# Autodesk Inventor assembly: joint4
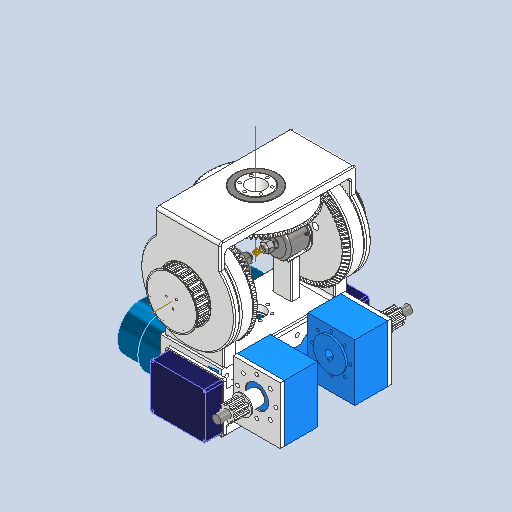
[picture p0: Inventor's stored thumbnail of the model, 512x512]
Saved by Autodesk Inventor 2025.3 (Build 293356030, 356C)
## iProperties
Created: 2025-08-31
Part Number: joint4
Document SubType Name: Assembly
Designer: MSI
Mass: 17943.2 g
Surface Area: 11658.9 cm^2
Volume: 6898.44 cm^3
Density: 2.60106 g/cm^3
Author: MSI
## Documents named in this file (16)
- C:\Users\MSI\Desktop\Project\3. 로봇팔\Robot Arm Model\Robot_Arm_6_v1\joint3.iam
- C:\Users\MSI\Desktop\Project\3. 로봇팔\Robot Arm Model\Robot_Arm_6_v1\base.ipt
- C:\Users\MSI\Desktop\Project\3. 로봇팔\Robot Arm Model\Robot_Arm_6_v1\frame.ipt
- C:\Users\MSI\Desktop\Project\3. 로봇팔\Robot Arm Model\Robot_Arm_6_v1\miter_gear_center.ipt
- C:\Users\MSI\Desktop\Project\3. 로봇팔\Robot Arm Model\Robot_Arm_6_v1\encoder.ipt
- C:\Users\MSI\Desktop\Project\3. 로봇팔\Robot Arm Model\Robot_Arm_6_v1\joint3_meteor.iam
- C:\Users\MSI\Desktop\Project\3. 로봇팔\Robot Arm Model\Robot_Arm_6_v1\encoder_frame.ipt
- C:\Users\MSI\Desktop\Project\3. 로봇팔\Robot Arm Model\Robot_Arm_6_v1\miter_gear_left_axis.ipt
- C:\Users\MSI\Desktop\Project\3. 로봇팔\Robot Arm Model\Robot_Arm_6_v1\miter_gear_right_axis.ipt
- C:\Users\MSI\Desktop\Project\3. 로봇팔\Robot Arm Model\Robot_Arm_6_v1\motor.iam
- C:\Users\MSI\Desktop\Project\3. 로봇팔\Robot Arm Model\Robot_Arm_6_v1\C-E6700ZZ_Autodesk_Inventor_2024_20250921\C-E6700ZZ.ipt
- C:\Users\MSI\Desktop\Project\3. 로봇팔\Robot Arm Model\Robot_Arm_6_v1\C-E6810ZZ_Autodesk_Inventor_2024_20250921\C-E6810ZZ.ipt
- C:\Users\MSI\Desktop\Project\3. 로봇팔\Robot Arm Model\Robot_Arm_6_v1\NTN_GS81110OuterRings\GS81110Outer Rings.ipt
- C:\Users\MSI\Desktop\Project\3. 로봇팔\Robot Arm Model\Robot_Arm_6_v1\belt_axis.ipt
- C:\Users\MSI\Desktop\Project\3. 로봇팔\Robot Arm Model\Robot_Arm_6_v1\joint3_belt_pulley_2.ipt
- C:\Users\MSI\Desktop\Project\3. 로봇팔\Robot Arm Model\Robot_Arm_6_v1\joint3_belt_pulley_1.ipt
## Components (23 placed, 14 different names)
1. motor:1 [sub-assembly] — 강체:24, 강체:36, 강체:37
2. base:1 — 회전:1, 강체:17, 강체:19, 강체:24, 강체:25, 강체:26
3. frame:1 — 회전:1, 회전:4, 강체:27, 강체:28, 강체:29, 강체:30, 강체:31
4. 베벨 기어2:1 — 회전:4
5. 베벨 기어1:3 — 강체:20
6. 베벨 기어1:4 — 강체:21
7. encoder:1 — 강체:18
8. encoder:2 — 강체:16
9. 동기식 풀리1:3 — 강체:36
10. 동기식 풀리1:4 — 강체:37
11. 동기식 풀리2:2 — 강체:35
12. 동기식 풀리2:1 — 강체:34
13. belt_axis:2 — 강체:33, 강체:35
14. belt_axis:1 — 강체:32, 강체:34
15. joint3_meteor:1 [sub-assembly] — 강체:20, 강체:25
16. joint3_meteor:2 [sub-assembly] — 강체:21, 강체:26
17. encoder_frame:1 — 강체:16, 강체:17
18. encoder_frame:2 — 강체:18, 강체:19
19. C-E6700ZZ:1 — 강체:27, 강체:32
20. C-E6700ZZ:2 — 강체:28, 강체:33
21. C-E6810ZZ:1 — 강체:29
22. GS81110Outer Rings:1 — 강체:30
23. GS81110Outer Rings:2 — 강체:31
## Relationships (22: WeldJoint 20, RevoluteJoint 2)
- 회전:1 [RevoluteJoint] (-1 mm): base:1 ↔ frame:1
- 회전:4 [RevoluteJoint] (-1 mm): frame:1 ↔ 베벨 기어2:1
- 강체:18 [WeldJoint]: encoder:1 ↔ encoder_frame:2
- 강체:16 [WeldJoint]: encoder:2 ↔ encoder_frame:1
- 강체:17 [WeldJoint]: base:1 ↔ encoder_frame:1
- 강체:19 [WeldJoint]: base:1 ↔ encoder_frame:2
- 강체:20 [WeldJoint] (2 mm): 베벨 기어1:3 ↔ joint3_meteor:1
- 강체:21 [WeldJoint] (-2 mm): 베벨 기어1:4 ↔ joint3_meteor:2
- 강체:24 [WeldJoint]: motor:1 ↔ base:1
- 강체:25 [WeldJoint]: base:1 ↔ joint3_meteor:1
- 강체:26 [WeldJoint]: base:1 ↔ joint3_meteor:2
- 강체:27 [WeldJoint]: frame:1 ↔ C-E6700ZZ:1
- 강체:28 [WeldJoint]: frame:1 ↔ C-E6700ZZ:2
- 강체:29 [WeldJoint] (-1 mm): frame:1 ↔ C-E6810ZZ:1
- 강체:30 [WeldJoint]: frame:1 ↔ GS81110Outer Rings:1
- 강체:31 [WeldJoint]: frame:1 ↔ GS81110Outer Rings:2
- 강체:32 [WeldJoint]: belt_axis:1 ↔ C-E6700ZZ:1
- 강체:33 [WeldJoint]: belt_axis:2 ↔ C-E6700ZZ:2
- 강체:34 [WeldJoint]: 동기식 풀리2:1 ↔ belt_axis:1
- 강체:35 [WeldJoint]: 동기식 풀리2:2 ↔ belt_axis:2
- 강체:36 [WeldJoint]: motor:1 ↔ 동기식 풀리1:3
- 강체:37 [WeldJoint]: motor:1 ↔ 동기식 풀리1:4
